# Autodesk Inventor assembly: 二輪足回り
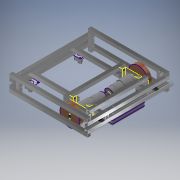
[picture p0: Inventor's stored thumbnail of the model, 180x180]
Saved by Autodesk Inventor 2018 (Build 220112000, 112)
## iProperties
Created: 2019-04-22
Part Number: 二輪足回り
Material: 一般
Document SubType Name: Assembly
Designer: Eiji Nishizawa
Author: Eiji Nishizawa
## Documents named in this file (18)
- G:\OneDrive\CAD\二輪足回り\二輪足回り.iam
- G:\OneDrive\CAD\二輪足回り\モーター100：1.iam
- G:\OneDrive\CAD\二輪足回り\モーターパーツ１.ipt
- G:\OneDrive\CAD\二輪足回り\モーターパーツ３.ipt
- G:\OneDrive\CAD\二輪足回り\モーターパーツ２.ipt
- G:\OneDrive\CAD\二輪足回り\スリットカラー.ipt
- G:\OneDrive\CAD\二輪足回り\タイヤ.ipt
- G:\OneDrive\CAD\二輪足回り\flontparts1.ipt
- G:\OneDrive\CAD\二輪足回り\backparts1.ipt
- G:\OneDrive\CAD\二輪足回り\f&bparts.ipt
- G:\OneDrive\CAD\二輪足回り\sideparts.ipt
- G:\OneDrive\CAD\二輪足回り\キャスター.ipt
- G:\OneDrive\CAD\二輪足回り\角パーツ.ipt
- G:\OneDrive\CAD\2018高専ロボコン\光センサー\光センサーケース.iam
- G:\OneDrive\CAD\二輪足回り\fsparts.ipt
- G:\OneDrive\CAD\二輪足回り\banperparts1.ipt
- G:\OneDrive\CAD\二輪足回り\banperparts2.ipt
- G:\OneDrive\CAD\二輪足回り\banper.ipt
## Components (38 placed, 17 different names)
1. モーター100：1:1 [sub-assembly] — 挿入:9, 挿入:10, 挿入:11, 挿入:12, 挿入:13, 挿入:14, 挿入:39
2. モーター100：1:2 [sub-assembly] — メイト:1, メイト:2, メイト:3, メイト:4, 挿入:27
3. モーターパーツ１:1 — 挿入:9, 挿入:10, 挿入:11, 挿入:12, 挿入:13, 挿入:14, 挿入:15, 挿入:16, 挿入:17, 挿入:18, 挿入:49, 挿入:50
4. モーターパーツ１:2 — メイト:1, メイト:2, メイト:3, メイト:4, 挿入:1, 挿入:2, 挿入:3, 挿入:4, 挿入:48, 挿入:51
5. モーターパーツ２:1 — 挿入:15, 挿入:16, 挿入:35
6. モーターパーツ２:2 — 挿入:17, 挿入:18, 挿入:31, 挿入:53
7. モーターパーツ２:3 — 挿入:3, 挿入:4, 挿入:32, 挿入:52
8. モーターパーツ２:4 — 挿入:1, 挿入:2, 挿入:36
9. スリットカラー:1 — 挿入:25, 挿入:26, 挿入:27
10. スリットカラー:2 — 挿入:37, 挿入:38, 挿入:39
11. タイヤ:1 — 挿入:25, 挿入:26
12. タイヤ:2 — 挿入:37, 挿入:38
13. flontparts1:1 — 挿入:32, 挿入:54, 挿入:80, 挿入:83, メイト:5, フラッシュ:2
14. flontparts1:2 — 挿入:31, 挿入:55, 挿入:81, 挿入:82, メイト:8
15. backparts1:1 — 挿入:36, 挿入:42
16. backparts1:2 — 挿入:35, 挿入:41
17. f&bparts:1 — 挿入:41, 挿入:42, 挿入:46, 挿入:47, 挿入:56, 挿入:57, 挿入:58, 挿入:59, 挿入:64, 挿入:65
18. sideparts:1 — 挿入:46, 挿入:61, 挿入:62, 挿入:84, 挿入:92
19. sideparts:2 — 挿入:47, 挿入:60, 挿入:63, 挿入:85, 挿入:93
20. モーターパーツ３:1 — 挿入:50, 挿入:51, 挿入:52, 挿入:53, 挿入:54, 挿入:55
21. モーターパーツ３:2 — 挿入:48, 挿入:49
22. キャスター:1 — 挿入:57, 挿入:58
23. キャスター:2 — 挿入:56, 挿入:59
24. 角パーツ:1 — 挿入:60, 挿入:74, 挿入:90, 挿入:91
25. 角パーツ:2 — 挿入:61, 挿入:75, 挿入:88, 挿入:89
26. 角パーツ:3 — 挿入:62, 挿入:65, 挿入:71, 挿入:76
27. 角パーツ:4 — 挿入:63, 挿入:64, 挿入:70, 挿入:77
28. f&bparts:3 — 挿入:70, 挿入:71, 挿入:78, 挿入:79
29. sideparts:3 — 挿入:75, 挿入:76, 挿入:79, 挿入:86, 挿入:94
30. sideparts:4 — 挿入:74, 挿入:77, 挿入:78, 挿入:87, 挿入:95
31. fsparts:1 — 挿入:80, 挿入:81, 挿入:84, 挿入:85, 挿入:88, 挿入:91, 挿入:92, 挿入:93, 挿入:96, 挿入:97, メイト:6, メイト:7
32. fsparts:2 — 挿入:82, 挿入:83, 挿入:86, 挿入:87, 挿入:89, 挿入:90, 挿入:94, 挿入:95, フラッシュ:1, フラッシュ:3, フラッシュ:6, フラッシュ:7
33. 光センサーケース:1 [sub-assembly] — 挿入:96, 挿入:97
34. banperparts1:1 — メイト:7, メイト:8, フラッシュ:3, メイト:11, メイト:12, フラッシュ:5
35. banperparts1:2 — メイト:5, フラッシュ:1, メイト:6, フラッシュ:2, メイト:9, メイト:10, フラッシュ:4
36. banperparts2:1 — メイト:9, メイト:10, フラッシュ:4, メイト:15, メイト:16
37. banperparts2:2 — メイト:11, メイト:12, フラッシュ:5, メイト:13, メイト:14
38. banper:1 — メイト:13, メイト:14, メイト:15, メイト:16, フラッシュ:6, フラッシュ:7
## Relationships (95: Insert 72, Mate 16, Flush 7)
- メイト:1 [Mate]: モーター100：1:2 ↔ モーターパーツ１:2
- メイト:2 [Mate]: モーター100：1:2 ↔ モーターパーツ１:2
- メイト:3 [Mate]: モーター100：1:2 ↔ モーターパーツ１:2
- メイト:4 [Mate]: モーター100：1:2 ↔ モーターパーツ１:2
- 挿入:1 [Insert]: モーターパーツ１:2 ↔ モーターパーツ２:4
- 挿入:2 [Insert]: モーターパーツ１:2 ↔ モーターパーツ２:4
- 挿入:3 [Insert]: モーターパーツ１:2 ↔ モーターパーツ２:3
- 挿入:4 [Insert]: モーターパーツ１:2 ↔ モーターパーツ２:3
- 挿入:9 [Insert]: モーター100：1:1 ↔ モーターパーツ１:1
- 挿入:10 [Insert]: モーター100：1:1 ↔ モーターパーツ１:1
- 挿入:11 [Insert]: モーター100：1:1 ↔ モーターパーツ１:1
- 挿入:12 [Insert]: モーター100：1:1 ↔ モーターパーツ１:1
- 挿入:13 [Insert]: モーター100：1:1 ↔ モーターパーツ１:1
- 挿入:14 [Insert]: モーター100：1:1 ↔ モーターパーツ１:1
- 挿入:15 [Insert]: モーターパーツ１:1 ↔ モーターパーツ２:1
- 挿入:16 [Insert]: モーターパーツ１:1 ↔ モーターパーツ２:1
- 挿入:17 [Insert]: モーターパーツ１:1 ↔ モーターパーツ２:2
- 挿入:18 [Insert]: モーターパーツ１:1 ↔ モーターパーツ２:2
- 挿入:25 [Insert]: スリットカラー:1 ↔ タイヤ:1
- 挿入:26 [Insert]: スリットカラー:1 ↔ タイヤ:1
- 挿入:27 [Insert]: モーター100：1:2 ↔ スリットカラー:1
- 挿入:31 [Insert]: モーターパーツ２:2 ↔ flontparts1:2
- 挿入:32 [Insert]: モーターパーツ２:3 ↔ flontparts1:1
- 挿入:35 [Insert]: モーターパーツ２:1 ↔ backparts1:2
- 挿入:36 [Insert]: モーターパーツ２:4 ↔ backparts1:1
- 挿入:37 [Insert]: スリットカラー:2 ↔ タイヤ:2
- 挿入:38 [Insert]: スリットカラー:2 ↔ タイヤ:2
- 挿入:39 [Insert]: モーター100：1:1 ↔ スリットカラー:2
- 挿入:41 [Insert]: backparts1:2 ↔ f&bparts:1
- 挿入:42 [Insert]: backparts1:1 ↔ f&bparts:1
- 挿入:46 [Insert]: f&bparts:1 ↔ sideparts:1
- 挿入:47 [Insert]: f&bparts:1 ↔ sideparts:2
- 挿入:48 [Insert]: モーターパーツ１:2 ↔ モーターパーツ３:2
- 挿入:49 [Insert]: モーターパーツ１:1 ↔ モーターパーツ３:2
- 挿入:50 [Insert]: モーターパーツ１:1 ↔ モーターパーツ３:1
- 挿入:51 [Insert]: モーターパーツ１:2 ↔ モーターパーツ３:1
- 挿入:52 [Insert]: モーターパーツ２:3 ↔ モーターパーツ３:1
- 挿入:53 [Insert]: モーターパーツ２:2 ↔ モーターパーツ３:1
- 挿入:54 [Insert]: flontparts1:1 ↔ モーターパーツ３:1
- 挿入:55 [Insert]: flontparts1:2 ↔ モーターパーツ３:1
- 挿入:56 [Insert]: f&bparts:1 ↔ キャスター:2
- 挿入:57 [Insert]: f&bparts:1 ↔ キャスター:1
- 挿入:58 [Insert]: f&bparts:1 ↔ キャスター:1
- 挿入:59 [Insert]: f&bparts:1 ↔ キャスター:2
- 挿入:60 [Insert]: sideparts:2 ↔ 角パーツ:1
- 挿入:61 [Insert]: sideparts:1 ↔ 角パーツ:2
- 挿入:62 [Insert]: sideparts:1 ↔ 角パーツ:3
- 挿入:63 [Insert]: sideparts:2 ↔ 角パーツ:4
- 挿入:64 [Insert]: f&bparts:1 ↔ 角パーツ:4
- 挿入:65 [Insert]: f&bparts:1 ↔ 角パーツ:3
- 挿入:70 [Insert]: 角パーツ:4 ↔ f&bparts:3
- 挿入:71 [Insert]: 角パーツ:3 ↔ f&bparts:3
- 挿入:74 [Insert]: 角パーツ:1 ↔ sideparts:4
- 挿入:75 [Insert]: 角パーツ:2 ↔ sideparts:3
- 挿入:76 [Insert]: 角パーツ:3 ↔ sideparts:3
- 挿入:77 [Insert]: 角パーツ:4 ↔ sideparts:4
- 挿入:78 [Insert]: f&bparts:3 ↔ sideparts:4
- 挿入:79 [Insert]: f&bparts:3 ↔ sideparts:3
- 挿入:80 [Insert]: flontparts1:1 ↔ fsparts:1
- 挿入:81 [Insert]: flontparts1:2 ↔ fsparts:1
- 挿入:82 [Insert]: flontparts1:2 ↔ fsparts:2
- 挿入:83 [Insert]: flontparts1:1 ↔ fsparts:2
- 挿入:84 [Insert]: sideparts:1 ↔ fsparts:1
- 挿入:85 [Insert]: sideparts:2 ↔ fsparts:1
- 挿入:86 [Insert]: sideparts:3 ↔ fsparts:2
- 挿入:87 [Insert]: sideparts:4 ↔ fsparts:2
- 挿入:88 [Insert]: 角パーツ:2 ↔ fsparts:1
- 挿入:89 [Insert]: 角パーツ:2 ↔ fsparts:2
- 挿入:90 [Insert]: 角パーツ:1 ↔ fsparts:2
- 挿入:91 [Insert]: 角パーツ:1 ↔ fsparts:1
- 挿入:92 [Insert]: sideparts:1 ↔ fsparts:1
- 挿入:93 [Insert]: sideparts:2 ↔ fsparts:1
- 挿入:94 [Insert]: sideparts:3 ↔ fsparts:2
- 挿入:95 [Insert]: sideparts:4 ↔ fsparts:2
- 挿入:96 [Insert]: fsparts:1 ↔ 光センサーケース:1
- 挿入:97 [Insert]: fsparts:1 ↔ 光センサーケース:1
- メイト:5 [Mate]: flontparts1:1 ↔ banperparts1:2
- フラッシュ:1 [Flush]: fsparts:2 ↔ banperparts1:2
- メイト:6 [Mate]: fsparts:1 ↔ banperparts1:2
- フラッシュ:2 [Flush]: flontparts1:1 ↔ banperparts1:2
- メイト:7 [Mate]: fsparts:1 ↔ banperparts1:1
- メイト:8 [Mate]: flontparts1:2 ↔ banperparts1:1
- フラッシュ:3 [Flush]: fsparts:2 ↔ banperparts1:1
- メイト:9 [Mate]: banperparts1:2 ↔ banperparts2:1
- メイト:10 [Mate]: banperparts1:2 ↔ banperparts2:1
- フラッシュ:4 [Flush]: banperparts1:2 ↔ banperparts2:1
- メイト:11 [Mate]: banperparts1:1 ↔ banperparts2:2
- メイト:12 [Mate]: banperparts1:1 ↔ banperparts2:2
- フラッシュ:5 [Flush]: banperparts1:1 ↔ banperparts2:2
- メイト:13 [Mate]: banperparts2:2 ↔ banper:1
- メイト:14 [Mate]: banperparts2:2 ↔ banper:1
- メイト:15 [Mate]: banperparts2:1 ↔ banper:1
- メイト:16 [Mate]: banperparts2:1 ↔ banper:1
- フラッシュ:6 [Flush]: fsparts:2 ↔ banper:1
- フラッシュ:7 [Flush]: fsparts:2 ↔ banper:1
